# Autodesk Inventor assembly: Extender
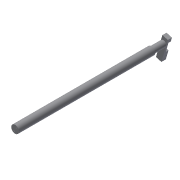
[picture p0: Inventor's stored thumbnail of the model, 180x180]
Saved by Autodesk Inventor 2015 (Build 190159000, 159)
## iProperties
Created: 2015-01-31
Part Number: Extender
Document SubType Name: Assembly
Designer: Tanner
Author: Tanner
## Documents named in this file (6)
- C:\Users\Noah\Desktop\FIRST-Team-1719-CAD-Team\2015 Robot CAD\Devices\Extender\Extender.iam
- C:\Users\Noah\Desktop\FIRST-Team-1719-CAD-Team\2015 Robot CAD\Devices\Extender\Tubing\Extender - .5 in tube.ipt
- C:\Users\Noah\Desktop\FIRST-Team-1719-CAD-Team\2015 Robot CAD\Devices\Extender\Tubing\Extender - .25 tube.ipt
- C:\Users\Noah\Desktop\FIRST-Team-1719-CAD-Team\2015 Robot CAD\Devices\Extender\Tubing\Extender - .75 in tube.ipt
- C:\Users\Noah\Desktop\FIRST-Team-1719-CAD-Team\2015 Robot CAD\Devices\Extender\Tubing\Extender - 1 in tube.ipt
- C:\Users\Noah\Desktop\FIRST-Team-1719-CAD-Team\2015 Robot CAD\Devices\Extender\Misc\Claw base.ipt
## Components (5 placed, 5 different names)
1. Extender - .5 in tube:1 — Mate:2, Mate:3, Flush:2, Flush:3
2. Extender - .25 tube:1 — Mate:3, Flush:3, Mate:4, Tangent:1, Tangent:2
3. Extender - .75 in tube:1 — Mate:1, Mate:2, Flush:1, Flush:2
4. Extender - 1 in tube:1 — Mate:1, Flush:1
5. Claw base:1 — Mate:4, Tangent:1, Tangent:2
## Relationships (9: Mate 4, Flush 3, Tangent 2)
- Mate:1: Extender - .75 in tube:1 ↔ Extender - 1 in tube:1
- Mate:2: Extender - .5 in tube:1 ↔ Extender - .75 in tube:1
- Mate:3: Extender - .5 in tube:1 ↔ Extender - .25 tube:1
- Flush:1: Extender - .75 in tube:1 ↔ Extender - 1 in tube:1
- Flush:2: Extender - .5 in tube:1 ↔ Extender - .75 in tube:1
- Flush:3: Extender - .5 in tube:1 ↔ Extender - .25 tube:1
- Mate:4: Extender - .25 tube:1 ↔ Claw base:1
- Tangent:1 (63.5 mm): Extender - .25 tube:1 ↔ Claw base:1
- Tangent:2 (4.1656 mm): Extender - .25 tube:1 ↔ Claw base:1
